# Autodesk Inventor assembly: Assembly1
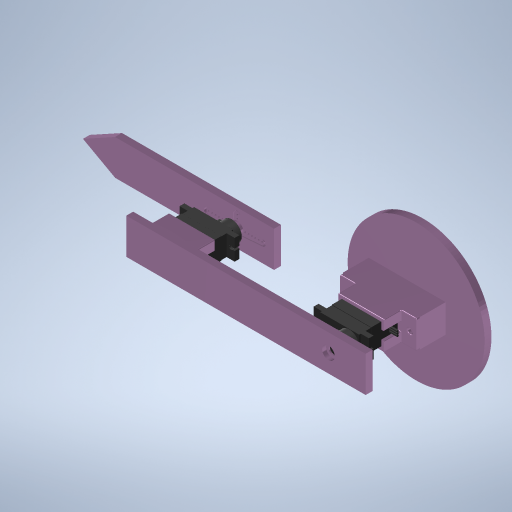
[picture p0: Inventor's stored thumbnail of the model, 512x512]
Saved by Autodesk Inventor 2023 (Build 270158000, 158)
## iProperties
Created: 2023-02-22
Part Number: Assembly1
Document SubType Name: Assembly
Designer: samue
Author: samue
## Documents named in this file (5)
- C:\Users\samue\Documents\Git\MatlabRaspy\Robot_Parts\Assembly1.iam
- C:\Users\samue\Documents\Git\MatlabRaspy\Robot_Parts\Base.ipt
- C:\Users\samue\Documents\Git\MatlabRaspy\Robot_Parts\ServoWithoutHorns.ipt
- C:\Users\samue\Documents\Git\MatlabRaspy\Robot_Parts\BackSegment_withHorns.ipt
- C:\Users\samue\Documents\Git\MatlabRaspy\Robot_Parts\FrontSegment_withHorns.ipt
## Components (5 placed, 4 different names)
1. Base:1 — Mate:1, Mate:2, Mate:3
2. ServoWithoutHorns:1 — Mate:1, Mate:2, Mate:3, Rotational:1
3. BackSegment_withHorns:1 — Rotational:1, Mate:4, Mate:5, Mate:6
4. ServoWithoutHorns:2 — Mate:4, Mate:5, Mate:6, Rotational:2
5. FrontSegment_withHorns:1 — Rotational:2
## Relationships (8: Mate 6, RevoluteJoint 2)
- Mate:1: Base:1 ↔ ServoWithoutHorns:1
- Mate:2: Base:1 ↔ ServoWithoutHorns:1
- Mate:3: Base:1 ↔ ServoWithoutHorns:1
- Rotational:1 [RevoluteJoint] (-76.2 mm): ServoWithoutHorns:1 ↔ BackSegment_withHorns:1
- Mate:4: BackSegment_withHorns:1 ↔ ServoWithoutHorns:2
- Mate:5: BackSegment_withHorns:1 ↔ ServoWithoutHorns:2
- Mate:6: BackSegment_withHorns:1 ↔ ServoWithoutHorns:2
- Rotational:2 [RevoluteJoint] (-76.2 mm): ServoWithoutHorns:2 ↔ FrontSegment_withHorns:1
## Named parameters: Simulation_Timeline = 0
